# Autodesk Inventor assembly: XMotor
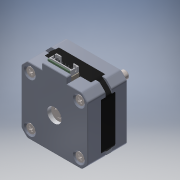
[picture p0: Inventor's stored thumbnail of the model, 180x180]
Saved by Autodesk Inventor 2019 (Build 230136000, 136)
## iProperties
Created: 2019-08-19
Part Number: XMotor
Document SubType Name: Assembly
Designer: Bruno
Author: Bruno
## Documents named in this file (3)
- C:\Users\Bruno\Stuff\Ajedrez2\XMotor.iam
- C:\Users\Bruno\Desktop\17HS10-0704S.ipt
- C:\Users\Bruno\Stuff\Ajedrez2\XMotorMount.ipt
## Components (2 placed, 2 different names)
1. 17HS10-0704S:1 — Rigid:1
2. XMotorMount:1 — Rigid:1
## Relationships (1: WeldJoint 1)
- Rigid:1 [WeldJoint]: 17HS10-0704S:1 ↔ XMotorMount:1
